# Autodesk Inventor assembly: talon stack
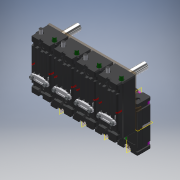
[picture p0: Inventor's stored thumbnail of the model, 180x180]
Saved by Autodesk Inventor 2019 (Build 230136000, 136)
## iProperties
Created: 2019-01-16
Part Number: talon stack
Document SubType Name: Assembly
Designer: pctech
Author: pctech
## Documents named in this file (5)
- T:\EIT\2019 Season\2019 ROBOT\COMMON PARTS\ELECTRONICS\VEX\talon stack.iam
- T:\EIT\2019 Season\2019 ROBOT\COMMON PARTS\ELECTRONICS\VEX\Talon_SRX_217-8080_No_Wires.ipt
- T:\EIT\2019 Season\2019 ROBOT\COMMON PARTS\ELECTRONICS\VEX\talon stack mount.ipt
- T:\EIT\2019 Season\2019 ROBOT\COMMON PARTS\ELECTRONICS\VEX\talon stack standoff.ipt
- T:\EIT\2019 Season\2019 ROBOT\COMMON PARTS\ELECTRONICS\VEX\Victor_SPX_217-9191.iam
## Components (11 placed, 4 different names)
1. talon stack mount:1 — Mate:1, Mate:2, Mate:3, Mate:4, Mate:5, Mate:6, Mate:15, Mate:16, Mate:17, Mate:18, Mate:19, Mate:20, Mate:21
2. Talon_SRX_217-8080_No_Wires:1 — Flush:3, Mate:6
3. Talon_SRX_217-8080_No_Wires:2 — Flush:1, Flush:2, Flush:3, Mate:4
4. Talon_SRX_217-8080_No_Wires:3 — Flush:2, Mate:1, Mate:2, Mate:3
5. Talon_SRX_217-8080_No_Wires:4 — Flush:1, Mate:5
6. Victor_SPX_217-9191:1 [sub-assembly] — Flush:5, Flush:6, Flush:9, Flush:12
7. Victor_SPX_217-9191:2 [sub-assembly] — Flush:5, Flush:8, Flush:9, Flush:10, Flush:12, Mate:19
8. Victor_SPX_217-9191:3 [sub-assembly] — Flush:4, Flush:7, Flush:11, Mate:20, Mate:21
9. Victor_SPX_217-9191:4 [sub-assembly] — Flush:4, Flush:6, Flush:7, Flush:8, Flush:10, Flush:11
10. talon stack standoff:1 — Mate:15, Mate:17
11. talon stack standoff:2 — Mate:16, Mate:18
## Relationships (25: Mate 13, Flush 12)
- Flush:1: Talon_SRX_217-8080_No_Wires:2 ↔ Talon_SRX_217-8080_No_Wires:4
- Flush:2: Talon_SRX_217-8080_No_Wires:2 ↔ Talon_SRX_217-8080_No_Wires:3
- Flush:3: Talon_SRX_217-8080_No_Wires:1 ↔ Talon_SRX_217-8080_No_Wires:2
- Mate:1: talon stack mount:1 ↔ Talon_SRX_217-8080_No_Wires:3
- Mate:2: talon stack mount:1 ↔ Talon_SRX_217-8080_No_Wires:3
- Mate:3: talon stack mount:1 ↔ Talon_SRX_217-8080_No_Wires:3
- Mate:4: talon stack mount:1 ↔ Talon_SRX_217-8080_No_Wires:2
- Mate:5: talon stack mount:1 ↔ Talon_SRX_217-8080_No_Wires:4
- Mate:6: talon stack mount:1 ↔ Talon_SRX_217-8080_No_Wires:1
- Mate:15: talon stack mount:1 ↔ talon stack standoff:1
- Mate:16: talon stack mount:1 ↔ talon stack standoff:2
- Mate:17: talon stack mount:1 ↔ talon stack standoff:1
- Mate:18: talon stack mount:1 ↔ talon stack standoff:2
- Flush:4: Victor_SPX_217-9191:3 ↔ Victor_SPX_217-9191:4
- Flush:5: Victor_SPX_217-9191:1 ↔ Victor_SPX_217-9191:2
- Flush:6: Victor_SPX_217-9191:1 ↔ Victor_SPX_217-9191:4
- Flush:7: Victor_SPX_217-9191:3 ↔ Victor_SPX_217-9191:4
- Flush:8: Victor_SPX_217-9191:2 ↔ Victor_SPX_217-9191:4
- Flush:9: Victor_SPX_217-9191:1 ↔ Victor_SPX_217-9191:2
- Flush:10 (31.75 mm): Victor_SPX_217-9191:2 ↔ Victor_SPX_217-9191:4
- Flush:11 (31.75 mm): Victor_SPX_217-9191:3 ↔ Victor_SPX_217-9191:4
- Flush:12 (31.75 mm): Victor_SPX_217-9191:1 ↔ Victor_SPX_217-9191:2
- Mate:19: talon stack mount:1 ↔ Victor_SPX_217-9191:2
- Mate:20: talon stack mount:1 ↔ Victor_SPX_217-9191:3
- Mate:21: talon stack mount:1 ↔ Victor_SPX_217-9191:3
